# Autodesk Inventor assembly: Rail_Assembly
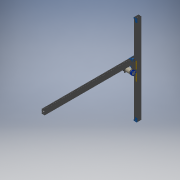
[picture p0: Inventor's stored thumbnail of the model, 180x180]
Saved by Autodesk Inventor 2019.4 (Build 234330000, 330)
## iProperties
Created: 2021-01-26
Part Number: Rail_Assembly
Document SubType Name: Assembly
Designer: Jorian Brusind
Mass: 3786.54 g
Surface Area: 19508.5 cm^2
Volume: 2323.9 cm^3
Density: 1.62939 g/cm^3
Author: Jorian Brusind
## Documents named in this file (11)
- C:\Users\Jorian Brusind\Documents\GitHub\PersonalProjects\HyperRail\Inventor Files\Rail_Assembly.iam
- C:\Users\Jorian Brusind\Documents\GitHub\PersonalProjects\Inventor Projects\Useful models\NEMA_Steppers\NEMA23\23HS8430B.ipt
- C:\Users\Jorian Brusind\Documents\GitHub\PersonalProjects\HyperRail\Inventor Files\NEMA23_StepperonlineMount.ipt
- C:\Users\Jorian Brusind\Documents\GitHub\PersonalProjects\HyperRail\Inventor Files\Roller_Bracket.iam
- C:\Users\Jorian Brusind\Documents\GitHub\PersonalProjects\HyperRail\Inventor Files\LargeBelt_Pulley.ipt
- C:\Users\Jorian Brusind\Documents\GitHub\PersonalProjects\Inventor Projects\Useful models\8020_Sets\IPT_40_Series\Extra_40_Series\HFS5-4060-4000\HFS5-4060-1275.ipt
- C:\Users\Jorian Brusind\Documents\GitHub\PersonalProjects\Inventor Projects\Useful models\8020_Sets\IPT_20_Series\IPT_20_Series\20-2040_200mm.ipt
- C:\Users\Jorian Brusind\Documents\GitHub\PersonalProjects\HyperRail\Inventor Files\2804S_NEMA2115_1Gearbox.ipt
- C:\Users\Jorian Brusind\Documents\GitHub\PersonalProjects\Inventor Projects\Useful models\8020_Sets\IPT_20_Series\Extra_20_Series\8020_14057m\14057_m.ipt
- C:\Users\Jorian Brusind\Documents\GitHub\PersonalProjects\HyperRail\Inventor Files\Large_Belt.ipt
- C:\Users\Jorian Brusind\Documents\GitHub\PersonalProjects\HyperRail\Inventor Files\Belt_Clamp.ipt
## Components (19 placed, 10 different names)
1. 23HS8430B:1 — Mate:18, Mate:23, Mate:24, Angle:1, Mate:48
2. NEMA23_StepperonlineMount:1 — Mate:18, Mate:23, Mate:24, Angle:1, Angle:2, Mate:49, Mate:57, Flush:14, Mate:59, Flush:15, Mate:61, Flush:16
3. Roller_Bracket:1 [sub-assembly] — Mate:78, Flush:29, Flush:31, Flush:32, Mate:81
4. Roller_Bracket:2 [sub-assembly] — Mate:79, Flush:30, Mate:80, Flush:31, Flush:32
5. LargeBelt_Pulley:1 — Mate:50, Mate:51, Flush:20, Mate:74, Mate:75
6. HFS5-4060-1275:1 — Flush:20, Mate:70, Flush:22, Mate:71, Mate:72, Flush:23, Mate:73, Flush:24, Mate:76, Flush:25, Flush:26, Mate:77, Flush:27, Flush:28, Mate:80, Mate:81
7. HFS5-4060-1275:2 — Flush:10, Mate:53, Mate:54, Mate:56, Mate:57, Flush:14, Mate:60, Mate:62, Mate:63, Mate:65, Flush:19
8. 20-2040_200mm:1 — Flush:10, Mate:52, Flush:12, Mate:55, Flush:13, Mate:56, Flush:17, Mate:64, Flush:18, Mate:66, Mate:78, Flush:29, Mate:79, Flush:30
9. 2804S_NEMA2115_1Gearbox:1 — Mate:48, Angle:2, Mate:49, Mate:50, Mate:51
10. 14057_m:1 — Mate:52, Flush:12, Mate:53, Flush:17
11. 14057_m:2 — Mate:54, Mate:55, Flush:13
12. 14057_m:3 — Mate:61, Mate:62, Flush:16
13. 14057_m:4 — Mate:59, Mate:60, Flush:15
14. 14057_m:5 — Mate:63, Mate:64, Flush:18
15. 14057_m:6 — Mate:65, Mate:66, Flush:19
16. Large_Belt:1 — Mate:72, Flush:23, Mate:75
17. Large_Belt:2 — Mate:73, Flush:24, Mate:74
18. Belt_Clamp:1 — Mate:76, Flush:25, Flush:26
19. Belt_Clamp:2 — Mate:77, Flush:27, Flush:28
## Relationships (56: Mate 33, Flush 21, Angle 2)
- Mate:18: 23HS8430B:1 ↔ NEMA23_StepperonlineMount:1
- Mate:23: 23HS8430B:1 ↔ NEMA23_StepperonlineMount:1
- Mate:24: 23HS8430B:1 ↔ NEMA23_StepperonlineMount:1
- Angle:1 (0 deg): 23HS8430B:1 ↔ NEMA23_StepperonlineMount:1
- Flush:10: HFS5-4060-1275:2 ↔ 20-2040_200mm:1
- Mate:48: 23HS8430B:1 ↔ 2804S_NEMA2115_1Gearbox:1
- Angle:2 (0 deg): NEMA23_StepperonlineMount:1 ↔ 2804S_NEMA2115_1Gearbox:1
- Mate:49: NEMA23_StepperonlineMount:1 ↔ 2804S_NEMA2115_1Gearbox:1
- Mate:50: LargeBelt_Pulley:1 ↔ 2804S_NEMA2115_1Gearbox:1
- Mate:51 (3 mm): LargeBelt_Pulley:1 ↔ 2804S_NEMA2115_1Gearbox:1
- Mate:52: 20-2040_200mm:1 ↔ 14057_m:1
- Flush:12: 20-2040_200mm:1 ↔ 14057_m:1
- Mate:53: HFS5-4060-1275:2 ↔ 14057_m:1
- Mate:54: HFS5-4060-1275:2 ↔ 14057_m:2
- Mate:55: 20-2040_200mm:1 ↔ 14057_m:2
- Flush:13: 20-2040_200mm:1 ↔ 14057_m:2
- Mate:56: HFS5-4060-1275:2 ↔ 20-2040_200mm:1
- Mate:57: NEMA23_StepperonlineMount:1 ↔ HFS5-4060-1275:2
- Flush:14 (-51.5 mm): NEMA23_StepperonlineMount:1 ↔ HFS5-4060-1275:2
- Mate:59: NEMA23_StepperonlineMount:1 ↔ 14057_m:4
- Mate:60: HFS5-4060-1275:2 ↔ 14057_m:4
- Flush:15: NEMA23_StepperonlineMount:1 ↔ 14057_m:4
- Mate:61: NEMA23_StepperonlineMount:1 ↔ 14057_m:3
- Mate:62: HFS5-4060-1275:2 ↔ 14057_m:3
- Flush:16: NEMA23_StepperonlineMount:1 ↔ 14057_m:3
- Flush:17: 20-2040_200mm:1 ↔ 14057_m:1
- Mate:63: HFS5-4060-1275:2 ↔ 14057_m:5
- Mate:64: 20-2040_200mm:1 ↔ 14057_m:5
- Flush:18: 20-2040_200mm:1 ↔ 14057_m:5
- Mate:65: HFS5-4060-1275:2 ↔ 14057_m:6
- Mate:66: 20-2040_200mm:1 ↔ 14057_m:6
- Flush:19: HFS5-4060-1275:2 ↔ 14057_m:6
- Flush:20: LargeBelt_Pulley:1 ↔ HFS5-4060-1275:1
- Mate:70: HFS5-4060-1275:1
- Flush:22: HFS5-4060-1275:1
- Mate:71: HFS5-4060-1275:1
- Mate:72: HFS5-4060-1275:1 ↔ Large_Belt:1
- Flush:23: HFS5-4060-1275:1 ↔ Large_Belt:1
- Mate:73: HFS5-4060-1275:1 ↔ Large_Belt:2
- Flush:24: HFS5-4060-1275:1 ↔ Large_Belt:2
- Mate:74 (25 mm): LargeBelt_Pulley:1 ↔ Large_Belt:2
- Mate:75 (25 mm): LargeBelt_Pulley:1 ↔ Large_Belt:1
- Mate:76: HFS5-4060-1275:1 ↔ Belt_Clamp:1
- Flush:25 (-2.5 mm): HFS5-4060-1275:1 ↔ Belt_Clamp:1
- Flush:26: HFS5-4060-1275:1 ↔ Belt_Clamp:1
- Mate:77: HFS5-4060-1275:1 ↔ Belt_Clamp:2
- Flush:27 (-2.5 mm): HFS5-4060-1275:1 ↔ Belt_Clamp:2
- Flush:28: HFS5-4060-1275:1 ↔ Belt_Clamp:2
- Mate:78: Roller_Bracket:1 ↔ 20-2040_200mm:1
- Flush:29: Roller_Bracket:1 ↔ 20-2040_200mm:1
- Mate:79: Roller_Bracket:2 ↔ 20-2040_200mm:1
- Flush:30: Roller_Bracket:2 ↔ 20-2040_200mm:1
- Mate:80: Roller_Bracket:2 ↔ HFS5-4060-1275:1
- Flush:31: Roller_Bracket:1 ↔ Roller_Bracket:2
- Flush:32: Roller_Bracket:1 ↔ Roller_Bracket:2
- Mate:81 (7 mm): Roller_Bracket:1 ↔ HFS5-4060-1275:1
